# Autodesk Inventor assembly: Assembly1
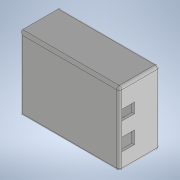
[picture p0: Inventor's stored thumbnail of the model, 180x180]
Saved by Autodesk Inventor 2020 (Build 240168000, 168)
## iProperties
Created: 2019-09-30
Part Number: Assembly1
Document SubType Name: Assembly
Designer: bzs3334
Author: bzs3334
## Documents named in this file (3)
- P:\LaserGazer\Assembly1.iam
- P:\LaserGazer\Case.ipt
- P:\LaserGazer\Lid.ipt
## Components (2 placed, 2 different names)
1. Case:1 — Mate:1, Mate:2, Mate:3, Mate:4, Mate:5
2. Lid:1 — Mate:1, Mate:2
## Relationships (5: Mate 5)
- Mate:1: Case:1 ↔ Lid:1
- Mate:2: Case:1 ↔ Lid:1
- Mate:3: Case:1
- Mate:4: Case:1
- Mate:5: Case:1
